# Autodesk Inventor assembly: booth
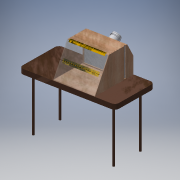
[picture p0: Inventor's stored thumbnail of the model, 180x180]
Saved by Autodesk Inventor 2017 (Build 210142000, 142)
## iProperties
Created: 2019-04-11
Part Number: booth
Document SubType Name: Assembly
Designer: Brian
Author: Brian
## Documents named in this file (23)
- B:\Miniatures\spray booth\booth.iam
- B:\Miniatures\spray booth\Frame - Horizontal (Bottom Front).ipt
- B:\Miniatures\spray booth\Frame - Horizontal (Bottom Rear).ipt
- B:\Miniatures\spray booth\Frame - Horizontal (Top Front).ipt
- B:\Miniatures\spray booth\Frame - Horizontal (Top Rear).ipt
- B:\Miniatures\spray booth\Back Side.ipt
- B:\Miniatures\spray booth\Cap Side.ipt
- B:\Miniatures\spray booth\Frame - Vertical (Clones).ipt
- B:\Miniatures\spray booth\Frame - Vertical (Left Front).ipt
- B:\Miniatures\spray booth\Top Side.ipt
- B:\Miniatures\spray booth\Left Side.ipt
- B:\Miniatures\spray booth\Bottom Base.ipt
- B:\Miniatures\spray booth\Right Side - Rear.ipt
- B:\Miniatures\spray booth\Right Side - Forward.ipt
- B:\Miniatures\spray booth\Filter.ipt
- B:\Miniatures\spray booth\Acrylic Panel - Top.ipt
- B:\Miniatures\spray booth\Acrylic Panel - Bottom.ipt
- B:\Miniatures\spray booth\PianoHingePlate.ipt
- B:\Miniatures\spray booth\dayton1TDT2 $167.ipt
- B:\Miniatures\spray booth\table.ipt
- B:\Miniatures\spray booth\attwood 4000.iam
- B:\Miniatures\spray booth\textures\Wrinkled Paper.jpg
- B:\Miniatures\spray booth\textures\images.png
## Components (23 placed, 20 different names)
1. Frame - Horizontal (Bottom Front):1 — Slider:1
2. Frame - Horizontal (Bottom Rear):1
3. Frame - Horizontal (Top Front):1
4. Frame - Horizontal (Top Rear):1
5. Back Side:1
6. Cap Side:1 — Rigid:2
7. Frame - Vertical (Clones):1
8. Frame - Vertical (Left Front):1
9. Top Side:1 — Mate:2
10. Left Side:1
11. Bottom Base:1 — Slider:2, Rigid:1
12. Right Side - Rear:1
13. Right Side - Forward:1 — Mate:4, Mate:9
14. Filter:1 — Slider:1
15. Acrylic Panel - Top:1 — Flush:1, Mate:7, Flush:9, Mate:10, Flush:2, Mate:11
16. Acrylic Panel - Bottom:1 — Mate:12, Flush:3, Mate:13
17. PianoHingePlate:1 — Flush:1, Mate:7, Flush:9, Rotational:1
18. PianoHingePlate:2 — Mate:2, Mate:4, Rotational:1, Mate:9
19. PianoHingePlate:3 — Mate:10, Flush:2, Mate:11, Rotational:2
20. PianoHingePlate:4 — Rotational:2, Mate:12, Flush:3, Mate:13
21. dayton1TDT2 $167:2 — Rigid:1
22. table:1 — Slider:2
23. attwood 4000:1 [sub-assembly] — Rigid:2
## Relationships (18: Mate 8, Flush 4, TranslationJoint 2, RevoluteJoint 2, WeldJoint 2)
- Slider:1 [TranslationJoint]: Frame - Horizontal (Bottom Front):1 ↔ Filter:1
- Mate:2: Top Side:1 ↔ PianoHingePlate:2
- Mate:4 (38.1 mm): Right Side - Forward:1 ↔ PianoHingePlate:2
- Flush:1 (38.1 mm): Acrylic Panel - Top:1 ↔ PianoHingePlate:1
- Mate:7: Acrylic Panel - Top:1 ↔ PianoHingePlate:1
- Flush:9 (-1.27 mm): Acrylic Panel - Top:1 ↔ PianoHingePlate:1
- Rotational:1 [RevoluteJoint]: PianoHingePlate:1 ↔ PianoHingePlate:2
- Mate:9 (6.35 mm): Right Side - Forward:1 ↔ PianoHingePlate:2
- Mate:10: Acrylic Panel - Top:1 ↔ PianoHingePlate:3
- Flush:2 (38.1 mm): Acrylic Panel - Top:1 ↔ PianoHingePlate:3
- Mate:11: Acrylic Panel - Top:1 ↔ PianoHingePlate:3
- Rotational:2 [RevoluteJoint]: PianoHingePlate:3 ↔ PianoHingePlate:4
- Mate:12: Acrylic Panel - Bottom:1 ↔ PianoHingePlate:4
- Flush:3 (38.1 mm): Acrylic Panel - Bottom:1 ↔ PianoHingePlate:4
- Mate:13: Acrylic Panel - Bottom:1 ↔ PianoHingePlate:4
- Slider:2 [TranslationJoint]: Bottom Base:1 ↔ table:1
- Rigid:1 [WeldJoint]: Bottom Base:1 ↔ dayton1TDT2 $167:2
- Rigid:2 [WeldJoint]: Cap Side:1 ↔ attwood 4000:1
